# Autodesk Inventor assembly: power supply
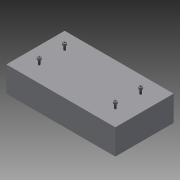
[picture p0: Inventor's stored thumbnail of the model, 180x180]
Saved by Autodesk Inventor 2013 (Build 170138000, 138)
## iProperties
Created: 2013-10-16
Part Number: power supply
Document SubType Name: Assembly
Designer: employee
Author: employee
## Documents named in this file (3)
- C:\Users\employee\Desktop\new wally\power supply.iam
- C:\Users\employee\Desktop\new wally\power supply.ipt
- C:\Users\employee\Desktop\new wally\M4x12.ipt
## Components (5 placed, 2 different names)
1. power supply:1 — Insert:1, Insert:2, Insert:3, Insert:4
2. Forged Socket Head Cap Screw - Metric M4x0.7 x 12:1 — Insert:1
3. Forged Socket Head Cap Screw - Metric M4x0.7 x 12:2 — Insert:4
4. Forged Socket Head Cap Screw - Metric M4x0.7 x 12:3 — Insert:3
5. Forged Socket Head Cap Screw - Metric M4x0.7 x 12:4 — Insert:2
## Relationships (4: Insert 4)
- Insert:1 (8.5 mm): power supply:1 ↔ Forged Socket Head Cap Screw - Metric M4x0.7 x 12:1
- Insert:2 (8.5 mm): power supply:1 ↔ Forged Socket Head Cap Screw - Metric M4x0.7 x 12:4
- Insert:3 (8.5 mm): power supply:1 ↔ Forged Socket Head Cap Screw - Metric M4x0.7 x 12:3
- Insert:4 (8.5 mm): power supply:1 ↔ Forged Socket Head Cap Screw - Metric M4x0.7 x 12:2
